# Autodesk Inventor assembly: spool double 2 in diameter
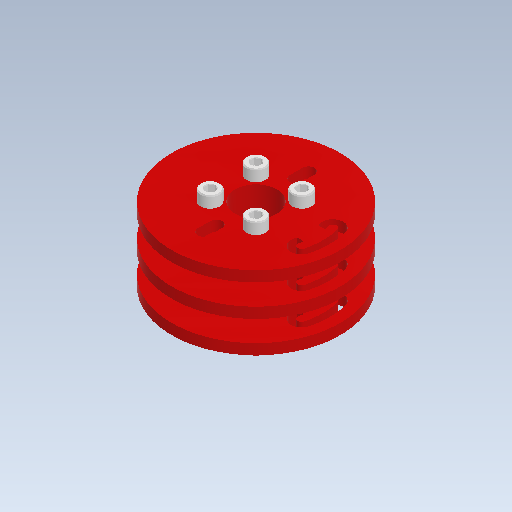
[picture p0: Inventor's stored thumbnail of the model, 512x512]
Saved by Autodesk Inventor 2020 (Build 240168000, 168)
## iProperties
Created: 2019-12-26
Part Number: spool double 2 in diameter
Document SubType Name: Assembly
Designer: ball
Author: ball
## Documents named in this file (5)
- D:\FTC8863\2019 Robot\Delivery\spool double 2 in diameter.iam
- D:\FTC8863\Actobotics\615 parts\615468 inner plate.ipt
- D:\FTC8863\Actobotics\615 parts\615468 outer plate 2_0 diameter.ipt
- D:\FTC8863\2019 Robot\Generic Parts\Clamping hub 6mm round shortened clamp.iam
- D:\FTC8863\StepLibraries\Screws\6-32 x 1.250 SOCKET HEAD CAP SCREW.ipt
## Components (12 placed, 4 different names)
1. 615468 inner plate:1 — Mate:1, Mate:2, Mate:3, Mate:4, Mate:5, Mate:6, Mate:10, Mate:11, Mate:12
2. 615468 inner plate:2 — Mate:3, Mate:4, Mate:5, Mate:6, Mate:7, Mate:8, Mate:9
3. 615468 outer plate 2_0 diameter:1 — Mate:7, Mate:8, Mate:9, Mate:26, Mate:28, Mate:30, Mate:32
4. 615468 outer plate 2_0 diameter:2 — Mate:10, Mate:11, Mate:12, Mate:20, Mate:21, Mate:22
5. 615468 inner plate:3
6. 615468 inner plate:4 — Mate:20, Mate:21, Mate:22
7. 615468 outer plate 2_0 diameter:3 — Mate:23, Mate:24, Mate:25
8. Clamping hub 6mm round shortened clamp:1 [sub-assembly] — Mate:23, Mate:24, Mate:25, Mate:27, Mate:29, Mate:31, Mate:33
9. 6-32 x 1.250 SOCKET HEAD CAP SCREW:1 — Mate:26, Mate:27
10. 6-32 x 1.250 SOCKET HEAD CAP SCREW:2 — Mate:30, Mate:31
11. 6-32 x 1.250 SOCKET HEAD CAP SCREW:3 — Mate:28, Mate:29
12. 6-32 x 1.250 SOCKET HEAD CAP SCREW:4 — Mate:32, Mate:33
## Relationships (33: Mate 33)
- Mate:1: 615468 inner plate:1
- Mate:2: 615468 inner plate:1
- Mate:3: 615468 inner plate:1 ↔ 615468 inner plate:2
- Mate:4: 615468 inner plate:1 ↔ 615468 inner plate:2
- Mate:5: 615468 inner plate:1 ↔ 615468 inner plate:2
- Mate:6: 615468 inner plate:1 ↔ 615468 inner plate:2
- Mate:7: 615468 inner plate:2 ↔ 615468 outer plate 2_0 diameter:1
- Mate:8: 615468 inner plate:2 ↔ 615468 outer plate 2_0 diameter:1
- Mate:9: 615468 inner plate:2 ↔ 615468 outer plate 2_0 diameter:1
- Mate:10: 615468 inner plate:1 ↔ 615468 outer plate 2_0 diameter:2
- Mate:11: 615468 inner plate:1 ↔ 615468 outer plate 2_0 diameter:2
- Mate:12: 615468 inner plate:1 ↔ 615468 outer plate 2_0 diameter:2
- [Mate]: 615468 inner plate:3 ↔ 615468 inner plate:4
- [Mate]: 615468 inner plate:3 ↔ 615468 inner plate:4
- [Mate]: 615468 inner plate:3 ↔ 615468 inner plate:4
- [Mate]: 615468 inner plate:3 ↔ 615468 inner plate:4
- [Mate]: 615468 inner plate:3 ↔ 615468 outer plate 2_0 diameter:3
- [Mate]: 615468 inner plate:3 ↔ 615468 outer plate 2_0 diameter:3
- [Mate]: 615468 inner plate:3 ↔ 615468 outer plate 2_0 diameter:3
- Mate:20: 615468 outer plate 2_0 diameter:2 ↔ 615468 inner plate:4
- Mate:21: 615468 outer plate 2_0 diameter:2 ↔ 615468 inner plate:4
- Mate:22: 615468 outer plate 2_0 diameter:2 ↔ 615468 inner plate:4
- Mate:23: 615468 outer plate 2_0 diameter:3 ↔ Clamping hub 6mm round shortened clamp:1
- Mate:24: 615468 outer plate 2_0 diameter:3 ↔ Clamping hub 6mm round shortened clamp:1
- Mate:25: 615468 outer plate 2_0 diameter:3 ↔ Clamping hub 6mm round shortened clamp:1
- Mate:26: 615468 outer plate 2_0 diameter:1 ↔ 6-32 x 1.250 SOCKET HEAD CAP SCREW:1
- Mate:27: Clamping hub 6mm round shortened clamp:1 ↔ 6-32 x 1.250 SOCKET HEAD CAP SCREW:1
- Mate:28: 615468 outer plate 2_0 diameter:1 ↔ 6-32 x 1.250 SOCKET HEAD CAP SCREW:3
- Mate:29: Clamping hub 6mm round shortened clamp:1 ↔ 6-32 x 1.250 SOCKET HEAD CAP SCREW:3
- Mate:30: 615468 outer plate 2_0 diameter:1 ↔ 6-32 x 1.250 SOCKET HEAD CAP SCREW:2
- Mate:31: Clamping hub 6mm round shortened clamp:1 ↔ 6-32 x 1.250 SOCKET HEAD CAP SCREW:2
- Mate:32: 615468 outer plate 2_0 diameter:1 ↔ 6-32 x 1.250 SOCKET HEAD CAP SCREW:4
- Mate:33: Clamping hub 6mm round shortened clamp:1 ↔ 6-32 x 1.250 SOCKET HEAD CAP SCREW:4
## Named parameters: d32_d30 = 0 mm, d33_d31 = 0 mm, d34_d22 = 0 mm, d35_d23 = 0 mm, d36_d24 = 0 mm, d37_d25 = 0 mm, d38_d29 = 0 mm
